# Autodesk Inventor assembly: two-section-bellows-on-bearings
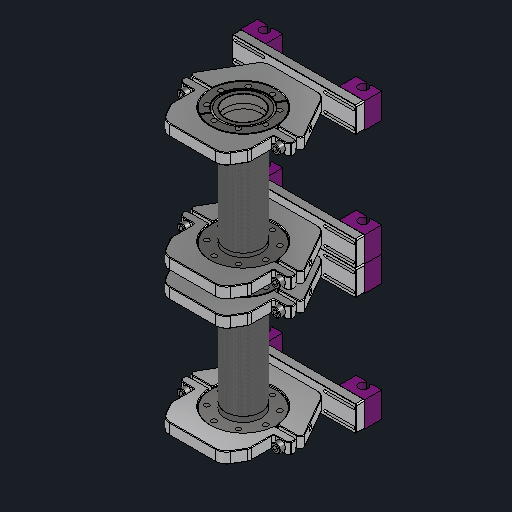
[picture p0: Inventor's stored thumbnail of the model, 512x512]
Saved by Autodesk Inventor 2027.1 (Build 311270010, 270A)
## iProperties
Part Number: two-section-bellows-on-bearings
Document SubType Name: Assembly
Designer: queezz
Author: queezz
## Documents named in this file (2)
- C:\Users\queezz\Dropbox\Drawings\pihti-cad\bellows-probe\two-section-bellows-on-bearings.iam
- C:\Users\queezz\Dropbox\Drawings\pihti-cad\bellows-probe\bellows-clamped-on-bearings.iam
## Components (2 placed, 1 different names)
1. bellows-clamped-on-bearings:1 [sub-assembly]
2. bellows-clamped-on-bearings:2 [sub-assembly]
## Relationships (1: Mate 1)
- [Mate]: bellows-clamped-on-bearings:1 ↔ bellows-clamped-on-bearings:2
